# Autodesk Inventor assembly: Link_1
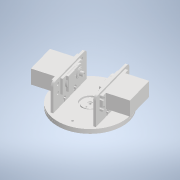
[picture p0: Inventor's stored thumbnail of the model, 180x180]
Saved by Autodesk Inventor 2022 (Build 260153000, 153)
## iProperties
Created: 2021-09-23
Part Number: Link_1
Document SubType Name: Assembly
Designer: Administrador
Author: Administrador
## Documents named in this file (6)
- C:\Users\Administrador\Desktop\Octavo Semestre\Robótica Industrial\Robot\Links\Link_1.iam
- C:\Users\Administrador\Desktop\Octavo Semestre\Robótica Industrial\Robot\Cuerpo\PartesCuerpo\Base3.ipt
- C:\Users\Administrador\Desktop\Octavo Semestre\Robótica Industrial\Robot\Cuerpo\PartesCuerpo\Circulo_Inferior.ipt
- C:\Users\Administrador\Desktop\Octavo Semestre\Robótica Industrial\Robot\Cuerpo\PartesCuerpo\Base4.ipt
- C:\Users\Administrador\Desktop\Octavo Semestre\Robótica Industrial\Robot\Cuerpo\PartesCuerpo\BaseMotoresHombrp.ipt
- C:\Users\Administrador\Desktop\Octavo Semestre\Robótica Industrial\Robot\Cuerpo\PartesCuerpo\Motor Mg995.ipt
## Components (6 placed, 5 different names)
1. Base3:1
2. Circulo_Inferior:1
3. Base4:1
4. BaseMotoresHombrp:1
5. Motor Mg995:1
6. Motor Mg995:2
## Relationships (16: Mate 15, WeldJoint 1)
- [Mate]: Base3:1 ↔ Circulo_Inferior:1
- [Mate]: Base3:1 ↔ Circulo_Inferior:1
- [Mate]: Base3:1 ↔ Circulo_Inferior:1
- [WeldJoint]: Base3:1 ↔ Circulo_Inferior:1
- [Mate]: Circulo_Inferior:1 ↔ Base4:1
- [Mate]: Base3:1 ↔ Base4:1
- [Mate]: Base3:1 ↔ Base4:1
- [Mate]: Base4:1 ↔ BaseMotoresHombrp:1
- [Mate]: Base4:1 ↔ BaseMotoresHombrp:1
- [Mate]: Base4:1 ↔ BaseMotoresHombrp:1
- [Mate]: BaseMotoresHombrp:1 ↔ Motor Mg995:1
- [Mate]: BaseMotoresHombrp:1 ↔ Motor Mg995:1
- [Mate]: BaseMotoresHombrp:1 ↔ Motor Mg995:1
- [Mate]: BaseMotoresHombrp:1 ↔ Motor Mg995:2
- [Mate]: BaseMotoresHombrp:1 ↔ Motor Mg995:2
- [Mate]: BaseMotoresHombrp:1 ↔ Motor Mg995:2
